# Autodesk Inventor assembly: Finger Assembly
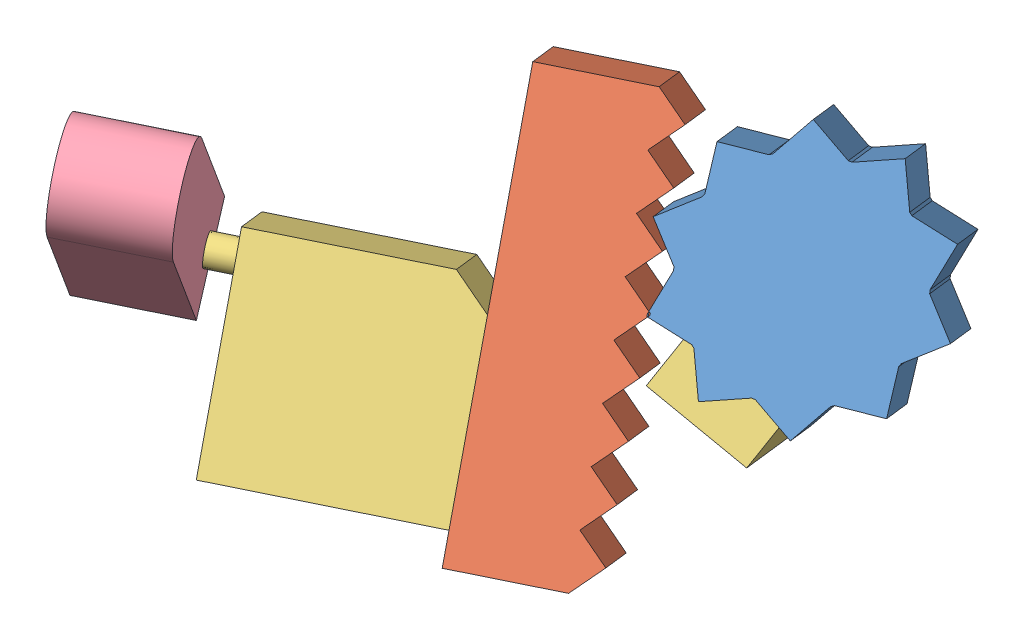
[picture p0: shaded view drawn from the shape stored in the file]
Saved by Autodesk Inventor 2023 (Build 270158000, 158)
## iProperties
Created: 2023-09-27
Part Number: Finger Assembly
Document SubType Name: Assembly
Designer: Turnt
Author: Turnt
## Documents named in this file (5)
- D:\School\ENEE408A\Modeling\Finger Assembly.iam
- D:\School\ENEE408A\Modeling\Finger Pinion.ipt
- D:\School\ENEE408A\Modeling\Finger Rack.ipt
- D:\School\ENEE408A\Modeling\Finger Servo.ipt
- D:\School\ENEE408A\Modeling\Finger.ipt
## Components (5 placed, 4 different names)
1. Finger Pinion:1 — Rotational:4, Flush:1
2. Finger Rack:1 — Rigid:1, Flush:1
3. Finger Servo:1 — Rigid:1, Rotational:3
4. Finger:1 — Rotational:3
5. Finger Servo:2 — Rotational:4
## Relationships (4: RevoluteJoint 2, WeldJoint 1, Flush 1)
- Rigid:1 [WeldJoint]: Finger Rack:1 ↔ Finger Servo:1
- Rotational:3 [RevoluteJoint]: Finger Servo:1 ↔ Finger:1
- Rotational:4 [RevoluteJoint] (2.54 mm): Finger Pinion:1 ↔ Finger Servo:2
- Flush:1: Finger Pinion:1 ↔ Finger Rack:1
